# Autodesk Inventor assembly: test assembly
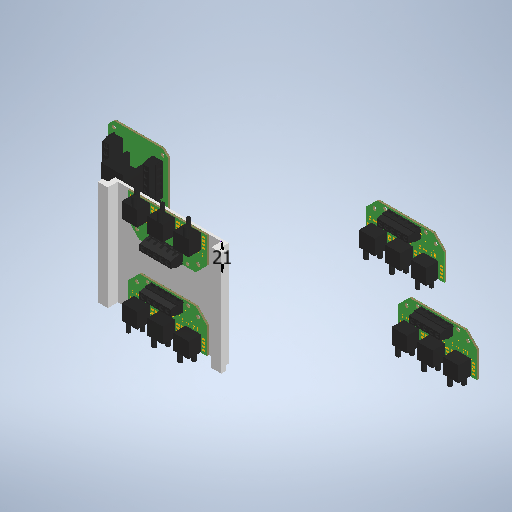
[picture p0: Inventor's stored thumbnail of the model, 512x512]
Saved by Autodesk Inventor 2025.1 (Build 291241000, 241)
## iProperties
Created: 2025-02-03
Part Number: test assembly
Document SubType Name: Assembly
Designer: johan
Author: johan
## Documents named in this file (4)
- C:\Users\johan\OneDrive - University of Bristol\CAD docs\2) Wing\Pressure tapping bits\test assembly.iam
- C:\Users\johan\OneDrive - University of Bristol\CAD docs\2) Wing\Avionics Cradle\Avionics Cradle (9-10).ipt
- C:\Users\johan\OneDrive - University of Bristol\CAD docs\2) Wing\Pressure tapping bits\PressureReadingBoard v4\PressureReadingBoard.iam
- C:\Users\johan\OneDrive - University of Bristol\CAD docs\2) Wing\Pressure tapping bits\Arduino Logger\Shield.iam
## Components (6 placed, 3 different names)
1. Avionics Cradle (9-10):1 — Rigid:1, Rigid:2
2. PressureReadingBoard:1 [sub-assembly]
3. PressureReadingBoard:2 [sub-assembly] — Rigid:1
4. PressureReadingBoard:3 [sub-assembly] — Rigid:2
5. PressureReadingBoard:4 [sub-assembly]
6. Shield:1 [sub-assembly]
## Relationships (2: WeldJoint 2)
- Rigid:1 [WeldJoint]: Avionics Cradle (9-10):1 ↔ PressureReadingBoard:2
- Rigid:2 [WeldJoint]: Avionics Cradle (9-10):1 ↔ PressureReadingBoard:3
